# Autodesk Inventor assembly: FrontHighBattery
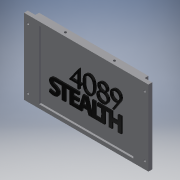
[picture p0: Inventor's stored thumbnail of the model, 180x180]
Saved by Autodesk Inventor 2019 (Build 230136000, 136)
## iProperties
Created: 2019-01-20
Part Number: FrontHighBattery
Document SubType Name: Assembly
Designer: james
Author: james
## Documents named in this file (4)
- F:\JimsDesign\2019CHS4089\FrontHighBattery.iam
- F:\JimsDesign\2019CHS4089\BatteryHighFront.ipt
- F:\JimsDesign\2019CHS4089\Stealth.ipt
- F:\JimsDesign\2019CHS4089\4089.ipt
## Components (3 placed, 3 different names)
1. BatteryHighFront:1 — Flush:1, Flush:2
2. Stealth:1 — Flush:1
3. 4089:1 — Flush:2
## Relationships (2: Flush 2)
- Flush:1: BatteryHighFront:1 ↔ Stealth:1
- Flush:2: BatteryHighFront:1 ↔ 4089:1
